# Autodesk Inventor assembly: s-assy-shooter_unit
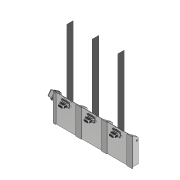
[picture p0: Inventor's stored thumbnail of the model, 180x180]
Saved by Autodesk Inventor 2022 (Build 260153000, 153)
## iProperties
Created: 2021-08-20
Part Number: s-assy-shooter_unit
Document SubType Name: Assembly
Designer: yuta0
Author: yuta0
## Documents named in this file (13)
- C:\Users\yuta0\Documents\GitHub\catchrobo_hardware\assy-shooter\s-assy-shooter_unit.iam
- C:\Users\yuta0\Documents\GitHub\catchrobo_hardware\assy-shooter\s_carbon_plate1.ipt
- C:\Users\yuta0\Documents\GitHub\catchrobo_hardware\assy-shooter\s_base2.ipt
- C:\Users\yuta0\Documents\GitHub\catchrobo_hardware\assy-shooter\s_base4.ipt
- C:\Users\yuta0\Downloads\新しいフォルダー\bisco.ipt
- C:\Users\yuta0\Documents\GitHub\catchrobo_hardware\assy-shooter\s-assy-guide_actuator.iam
- C:\Users\yuta0\Documents\GitHub\catchrobo_hardware\assy-shooter\MF126ZZ.ipt
- C:\Users\yuta0\Documents\GitHub\catchrobo_hardware\assy-shooter\s_shaft.ipt
- C:\Users\yuta0\Documents\GitHub\catchrobo_hardware\assy-shooter\CPRC16-6-6.iam
- C:\Users\yuta0\Documents\GitHub\catchrobo_hardware\assy-shooter\SCSTR6-8.iam
- C:\Users\yuta0\Documents\GitHub\catchrobo_hardware\assy-robot\CB4-10.ipt
- C:\Users\yuta0\Documents\GitHub\catchrobo_hardware\assy-shooter\s_carbon_plate5.ipt
- C:\Users\yuta0\Documents\GitHub\catchrobo_hardware\assy-shooter\s-assy-sorter.iam
## Components (28 placed, 12 different names)
1. s_base4:1 — メイト:20, メイト:21, フラッシュ:6, メイト:51, メイト:53, メイト:54, メイト:55, メイト:56, メイト:69, メイト:70, メイト:71, メイト:72, メイト:73, メイト:74, メイト:75, メイト:76, メイト:79
2. s-assy-guide_actuator:1 [sub-assembly] — メイト:51, メイト:63, メイト:69, メイト:70
3. MF126ZZ:1 — メイト:53, メイト:54, メイト:62
4. MF126ZZ:2 — メイト:55, メイト:56
5. MF126ZZ:3 — メイト:58, メイト:59
6. MF126ZZ:4 — メイト:60, メイト:61
7. s_shaft:1 — メイト:62, メイト:63, メイト:64, メイト:67, メイト:77, メイト:88, メイト:89
8. CPRC16-6-6:1 [sub-assembly] — メイト:64, メイト:65
9. CB4-10:1 — メイト:71, メイト:72
10. CB4-10:2 — メイト:73, メイト:74
11. CB4-10:3 — メイト:75, メイト:76
12. bisco:2 — メイト:84, メイト:85, 角度:2, 正接:1
13. s_shaft:2 — メイト:88, メイト:89
14. s-assy-sorter:1 [sub-assembly] — メイト:80, メイト:81, メイト:82
15. s_carbon_plate1:1 — メイト:13, メイト:14, メイト:20, メイト:21, フラッシュ:5, フラッシュ:6, メイト:80, メイト:81, メイト:82, 角度:1, メイト:84, 角度:2
16. s_base2:1 — メイト:13, メイト:14, フラッシュ:5, メイト:58, メイト:59, メイト:60, メイト:61, メイト:65, メイト:85
17. SCSTR6-8:1 [sub-assembly] — メイト:67, メイト:78, 正接:1
18. s_carbon_plate5:1 — メイト:77, メイト:78, メイト:79, 角度:1
19. s-assy-sorter:2 [sub-assembly]
20. s_carbon_plate1:2
21. s_base2:2
22. SCSTR6-8:3 [sub-assembly]
23. s_carbon_plate5:2
24. s-assy-sorter:3 [sub-assembly]
25. s_carbon_plate1:3
26. s_base2:3
27. SCSTR6-8:4 [sub-assembly]
28. s_carbon_plate5:3
## Component patterns: (3 elements, first: s-assy-sorter:1 + s_carbon_plate1:1 + s_base2:1 + SCSTR6-8:1 + s_carbon_plate5:1)
## Relationships (41: Mate 36, Flush 2, Angle 2, Tangent 1)
- メイト:13 [Mate]: s_carbon_plate1:1 ↔ s_base2:1
- メイト:14 [Mate]: s_carbon_plate1:1 ↔ s_base2:1
- メイト:20 [Mate]: s_base4:1 ↔ s_carbon_plate1:1
- メイト:21 [Mate]: s_base4:1 ↔ s_carbon_plate1:1
- フラッシュ:5 [Flush]: s_carbon_plate1:1 ↔ s_base2:1
- フラッシュ:6 [Flush]: s_base4:1 ↔ s_carbon_plate1:1
- メイト:51 [Mate]: s_base4:1 ↔ s-assy-guide_actuator:1
- メイト:53 [Mate]: s_base4:1 ↔ MF126ZZ:1
- メイト:54 [Mate]: s_base4:1 ↔ MF126ZZ:1
- メイト:55 [Mate]: s_base4:1 ↔ MF126ZZ:2
- メイト:56 [Mate]: s_base4:1 ↔ MF126ZZ:2
- メイト:58 [Mate]: MF126ZZ:3 ↔ s_base2:1
- メイト:59 [Mate]: MF126ZZ:3 ↔ s_base2:1
- メイト:60 [Mate]: MF126ZZ:4 ↔ s_base2:1
- メイト:61 [Mate]: MF126ZZ:4 ↔ s_base2:1
- メイト:62 [Mate]: MF126ZZ:1 ↔ s_shaft:1
- メイト:63 [Mate]: s-assy-guide_actuator:1 ↔ s_shaft:1
- メイト:64 [Mate]: s_shaft:1 ↔ CPRC16-6-6:1
- メイト:65 [Mate] (79.5 mm): CPRC16-6-6:1 ↔ s_base2:1
- メイト:67 [Mate]: s_shaft:1 ↔ SCSTR6-8:1
- メイト:69 [Mate]: s_base4:1 ↔ s-assy-guide_actuator:1
- メイト:70 [Mate]: s_base4:1 ↔ s-assy-guide_actuator:1
- メイト:71 [Mate]: s_base4:1 ↔ CB4-10:1
- メイト:72 [Mate]: s_base4:1 ↔ CB4-10:1
- メイト:73 [Mate]: s_base4:1 ↔ CB4-10:2
- メイト:74 [Mate]: s_base4:1 ↔ CB4-10:2
- メイト:75 [Mate]: s_base4:1 ↔ CB4-10:3
- メイト:76 [Mate]: s_base4:1 ↔ CB4-10:3
- メイト:77 [Mate]: s_shaft:1 ↔ s_carbon_plate5:1
- メイト:78 [Mate]: SCSTR6-8:1 ↔ s_carbon_plate5:1
- メイト:79 [Mate] (87.5 mm): s_base4:1 ↔ s_carbon_plate5:1
- メイト:80 [Mate]: s-assy-sorter:1 ↔ s_carbon_plate1:1
- メイト:81 [Mate]: s-assy-sorter:1 ↔ s_carbon_plate1:1
- メイト:82 [Mate]: s-assy-sorter:1 ↔ s_carbon_plate1:1
- 角度:1 [Angle] (0 deg): s_carbon_plate1:1 ↔ s_carbon_plate5:1
- メイト:84 [Mate]: bisco:2 ↔ s_carbon_plate1:1
- メイト:85 [Mate]: bisco:2 ↔ s_base2:1
- 角度:2 [Angle] (120 deg): bisco:2 ↔ s_carbon_plate1:1
- 正接:1 [Tangent] (30 mm): bisco:2 ↔ SCSTR6-8:1
- メイト:88 [Mate]: s_shaft:1 ↔ s_shaft:2
- メイト:89 [Mate]: s_shaft:1 ↔ s_shaft:2
